# Autodesk Inventor assembly: GE-12092
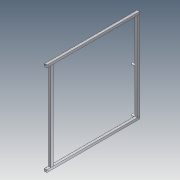
[picture p0: Inventor's stored thumbnail of the model, 180x180]
Saved by Autodesk Inventor 2012 (Build 160160000, 160)
## iProperties
Created: 2011-10-10
Part Number: GE-12092
Document SubType Name: Assembly
Designer: dfoster
Description: Corral Frame, Left
Title: Corral Frame, Left
Author: dfoster
## Documents named in this file (4)
- C:\Data Folder\FRC 2012 Field\Components\GE-12092.iam
- C:\Data Folder\FRC 2012 Field\Components\GE-12092-01.ipt
- C:\Data Folder\FRC 2012 Field\Components\GE-12092-02.ipt
- C:\Data Folder\FRC 2012 Field\Components\GE-12092-03.ipt
## Components (6 placed, 3 different names)
1. GE-12092-01:1 — Flush:5, Flush:1, Flush:3, Flush:2, Mate:1
2. GE-12092-01:2 — Flush:5, Flush:4, Mate:2
3. GE-12092-02:1 — Flush:1
4. GE-12092-02:2 — Flush:4, Mate:2, Flush:3, Flush:2, Mate:1
5. GE-12092-03:1
6. GE-12092-03:2
## Relationships (13: Mate 8, Flush 5)
- Flush:5: GE-12092-01:1 ↔ GE-12092-01:2
- Flush:1: GE-12092-01:1 ↔ GE-12092-02:1
- Flush:4: GE-12092-01:2 ↔ GE-12092-02:2
- Mate:2: GE-12092-01:2 ↔ GE-12092-02:2
- Flush:3 (50.8 mm): GE-12092-01:1 ↔ GE-12092-02:2
- Flush:2: GE-12092-01:1 ↔ GE-12092-02:2
- Mate:1: GE-12092-01:1 ↔ GE-12092-02:2
- [Mate] (-15.875 mm): GE-12092-01:1 ↔ GE-12092-03:1
- [Mate] (-15.875 mm): GE-12092-01:1 ↔ GE-12092-03:1
- [Mate] (-593.725 mm): GE-12092-01:1 ↔ GE-12092-03:2
- [Mate] (-15.875 mm): GE-12092-02:1 ↔ GE-12092-03:2
- [Mate]: GE-12092-01:1 ↔ GE-12092-03:1
- [Mate]: GE-12092-02:1 ↔ GE-12092-03:2
